# Autodesk Inventor assembly: Assembly_Cube_v4_KinematicMirror_45°
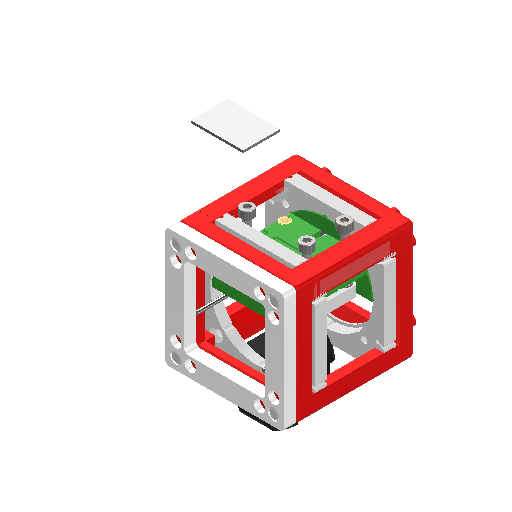
[picture p0: Inventor's stored thumbnail of the model, 512x512]
Saved by Autodesk Inventor 2025.1 (Build 291241020, 241B)
## iProperties
Created: 2024-10-03
Part Number: Assembly_Cube_v4_KinematicMirror_45°
Document SubType Name: Assembly
Designer: diederichbenedict
Author: diederichbenedict
## Documents named in this file (11)
- C:\Users\diederichbenedict\Dropbox\Dokumente\Promotion\PROJECTS\TechnicalDocs-openUC2-QBox\Production_Files\CAD_Files\INVENTOR\Assembly_Cube_v4_KinematicMirror_45°.iam
- C:\Users\diederichbenedict\Dropbox\Dokumente\Promotion\PROJECTS\TechnicalDocs-openUC2-QBox\Production_Files\CAD_Files\INVENTOR\Assembly_Cube_v4.iam
- C:\Users\diederichbenedict\Dropbox\Dokumente\Promotion\PROJECTS\TechnicalDocs-openUC2-QBox\Production_Files\CAD_Files\INVENTOR\10_Insert_v4.ipt
- C:\Users\diederichbenedict\Dropbox\Dokumente\Promotion\PROJECTS\TechnicalDocs-openUC2-QBox\Production_Files\CAD_Files\INVENTOR\20_Cube_4_insert_Lens_kinematic_mirrormount_45_90.ipt
- C:\Users\diederichbenedict\Dropbox\Dokumente\Promotion\PROJECTS\TechnicalDocs-openUC2-QBox\Production_Files\CAD_Files\INVENTOR\20_Cube_4_insert_Lens_kinematic_mirrormount_plate.ipt
- C:\Users\diederichbenedict\Dropbox\Dokumente\Promotion\PROJECTS\TechnicalDocs-openUC2-QBox\Production_Files\CAD_Files\INVENTOR\00_ruthex_RX-M3x4.0_SHORT\00_ruthex_RX-M3x4.0_SHORT\00_ruthex_RX-M3x4.0_SHORT.iam
- C:\Users\diederichbenedict\Dropbox\Dokumente\Promotion\PROJECTS\TechnicalDocs-openUC2-QBox\Production_Files\CAD_Files\INVENTOR\DIN 912 - M3 x 0.5 x 20 x 18.75.ipt
- C:\Users\diederichbenedict\Dropbox\Dokumente\Promotion\PROJECTS\TechnicalDocs-openUC2-QBox\Production_Files\CAD_Files\INVENTOR\00_Magnet_Neodym_5mm.ipt
- C:\Users\diederichbenedict\Dropbox\Dokumente\Promotion\PROJECTS\TechnicalDocs-openUC2-QBox\Production_Files\CAD_Files\INVENTOR\00_Mirror_astromedia_22x15.5.ipt
- C:\Users\diederichbenedict\Dropbox\Dokumente\Promotion\PROJECTS\TechnicalDocs-openUC2-QBox\Production_Files\CAD_Files\INVENTOR\00_3M_StickyPad.ipt
- C:\Users\diederichbenedict\Dropbox\Dokumente\Promotion\PROJECTS\TechnicalDocs-openUC2-QBox\Production_Files\CAD_Files\INVENTOR\00_kinematic_mirror_mount_SM05_taobao.ipt
## Components (20 placed, 10 different names)
1. Assembly_Cube_v4:1 [sub-assembly] — Mate:1, Mate:2, Mate:5, Angle:1, Mate:7
2. 20_Cube_4_insert_Lens_kinematic_mirrormount_45_90:1 — Flush:4, Angle:2, Flush:5, Insert:1, Insert:2, Flush:8, Mate:8, Mate:9, Insert:7
3. 20_Cube_4_insert_Lens_kinematic_mirrormount_plate:1 — Mate:10, Mate:11, Mate:12, Insert:9, Angle:3, Flush:9
4. 20_Cube_4_insert_Lens_kinematic_mirrormount_45_90:2 — Insert:3, Insert:4, Flush:8, Mate:8, Mate:9, Insert:8, Mate:13, Angle:3
5. 00_ruthex_RX-M3x4.0_SHORT:1 [sub-assembly] — Insert:3
6. 00_ruthex_RX-M3x4.0_SHORT:2 [sub-assembly] — Insert:1, Insert:6
7. 00_ruthex_RX-M3x4.0_SHORT:3 [sub-assembly] — Insert:2
8. 00_ruthex_RX-M3x4.0_SHORT:4 [sub-assembly] — Insert:4, Insert:5
9. DIN 912 - replaced by DIN EN ISO 4762 M3 x 20:1 — Insert:7
10. DIN 912 - replaced by DIN EN ISO 4762 M3 x 20:2 — Insert:6
11. DIN 912 - replaced by DIN EN ISO 4762 M3 x 20:3 — Insert:5, Insert:9
12. DIN 912 - replaced by DIN EN ISO 4762 M3 x 20:4 — Insert:8
13. 00_Magnet_Neodym_5mm:1 — Mate:10
14. 00_Magnet_Neodym_5mm:2 — Mate:11
15. 00_Magnet_Neodym_5mm:3 — Mate:12
16. 00_Mirror_astromedia_22x15.5:1 — Flush:9
17. 00_3M_StickyPad:1
18. 00_kinematic_mirror_mount_SM05_taobao:1
19. 10_Insert_v4:1 — Flush:4, Mate:5, Angle:1, Angle:2, Mate:7
20. 10_Insert_v4:2 — Flush:5, Mate:13
## Component patterns: (2 elements, first: 10_Insert_v4:1)
## Relationships (26: Mate 10, Insert 9, Flush 4, Angle 3)
- Mate:1: Assembly_Cube_v4:1
- Mate:2: Assembly_Cube_v4:1
- Flush:4: 20_Cube_4_insert_Lens_kinematic_mirrormount_45_90:1 ↔ 10_Insert_v4:1
- Mate:5: Assembly_Cube_v4:1 ↔ 10_Insert_v4:1
- Angle:1 (180 deg): Assembly_Cube_v4:1 ↔ 10_Insert_v4:1
- Angle:2 (180 deg): 20_Cube_4_insert_Lens_kinematic_mirrormount_45_90:1 ↔ 10_Insert_v4:1
- Mate:7: Assembly_Cube_v4:1 ↔ 10_Insert_v4:1
- Flush:5: 20_Cube_4_insert_Lens_kinematic_mirrormount_45_90:1 ↔ 10_Insert_v4:2
- Insert:1: 20_Cube_4_insert_Lens_kinematic_mirrormount_45_90:1 ↔ 00_ruthex_RX-M3x4.0_SHORT:2
- Insert:2: 20_Cube_4_insert_Lens_kinematic_mirrormount_45_90:1 ↔ 00_ruthex_RX-M3x4.0_SHORT:3
- Insert:3: 20_Cube_4_insert_Lens_kinematic_mirrormount_45_90:2 ↔ 00_ruthex_RX-M3x4.0_SHORT:1
- Insert:4: 20_Cube_4_insert_Lens_kinematic_mirrormount_45_90:2 ↔ 00_ruthex_RX-M3x4.0_SHORT:4
- Flush:8: 20_Cube_4_insert_Lens_kinematic_mirrormount_45_90:1 ↔ 20_Cube_4_insert_Lens_kinematic_mirrormount_45_90:2
- Mate:8: 20_Cube_4_insert_Lens_kinematic_mirrormount_45_90:1 ↔ 20_Cube_4_insert_Lens_kinematic_mirrormount_45_90:2
- Mate:9: 20_Cube_4_insert_Lens_kinematic_mirrormount_45_90:1 ↔ 20_Cube_4_insert_Lens_kinematic_mirrormount_45_90:2
- Insert:5 (-10 mm): 00_ruthex_RX-M3x4.0_SHORT:4 ↔ DIN 912 - replaced by DIN EN ISO 4762 M3 x 20:3
- Insert:6 (-10 mm): 00_ruthex_RX-M3x4.0_SHORT:2 ↔ DIN 912 - replaced by DIN EN ISO 4762 M3 x 20:2
- Insert:7 (-10 mm): 20_Cube_4_insert_Lens_kinematic_mirrormount_45_90:1 ↔ DIN 912 - replaced by DIN EN ISO 4762 M3 x 20:1
- Insert:8: 20_Cube_4_insert_Lens_kinematic_mirrormount_45_90:2 ↔ DIN 912 - replaced by DIN EN ISO 4762 M3 x 20:4
- Mate:10: 20_Cube_4_insert_Lens_kinematic_mirrormount_plate:1 ↔ 00_Magnet_Neodym_5mm:1
- Mate:11: 20_Cube_4_insert_Lens_kinematic_mirrormount_plate:1 ↔ 00_Magnet_Neodym_5mm:2
- Mate:12: 20_Cube_4_insert_Lens_kinematic_mirrormount_plate:1 ↔ 00_Magnet_Neodym_5mm:3
- Mate:13: 20_Cube_4_insert_Lens_kinematic_mirrormount_45_90:2 ↔ 10_Insert_v4:2
- Insert:9: 20_Cube_4_insert_Lens_kinematic_mirrormount_plate:1 ↔ DIN 912 - replaced by DIN EN ISO 4762 M3 x 20:3
- Angle:3 (90 deg): 20_Cube_4_insert_Lens_kinematic_mirrormount_plate:1 ↔ 20_Cube_4_insert_Lens_kinematic_mirrormount_45_90:2
- Flush:9: 20_Cube_4_insert_Lens_kinematic_mirrormount_plate:1 ↔ 00_Mirror_astromedia_22x15.5:1
